# Autodesk Inventor assembly: Limelight
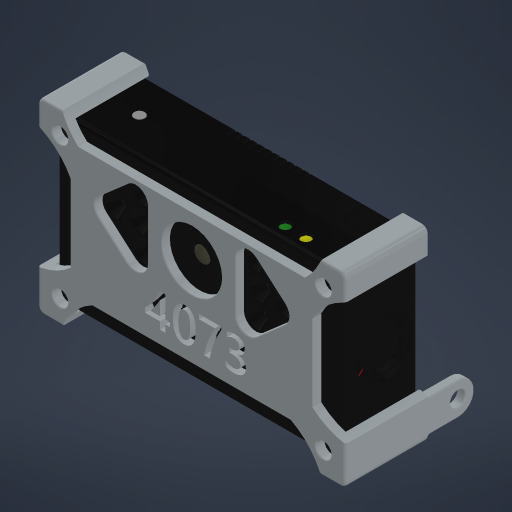
[picture p0: Inventor's stored thumbnail of the model, 512x512]
Saved by Autodesk Inventor 2023 (Build 270158000, 158)
## iProperties
Created: 2022-04-16
Part Number: Limelight
Document SubType Name: Assembly
Designer: timmy
Author: timmy
## Documents named in this file (3)
- R:\Inventor\RoboCatz\T-Shirt\Rev2-Better\Limelight.iam
- R:\Inventor\RoboCatz\T-Shirt\Rev2-Better\frc2020-limelight-box-1.snapshot.1\BOX.ipt
- R:\Inventor\RoboCatz\T-Shirt\Rev2-Better\Limelight.ipt
## Components (2 placed, 2 different names)
1. BOX:1 — Mate:1, Mate:2, Mate:3
2. Limelight:1 — Mate:1, Mate:2, Mate:3
## Relationships (3: Mate 3)
- Mate:1: BOX:1 ↔ Limelight:1
- Mate:2: BOX:1 ↔ Limelight:1
- Mate:3: BOX:1 ↔ Limelight:1
